# Autodesk Inventor assembly: ASM X-Axis
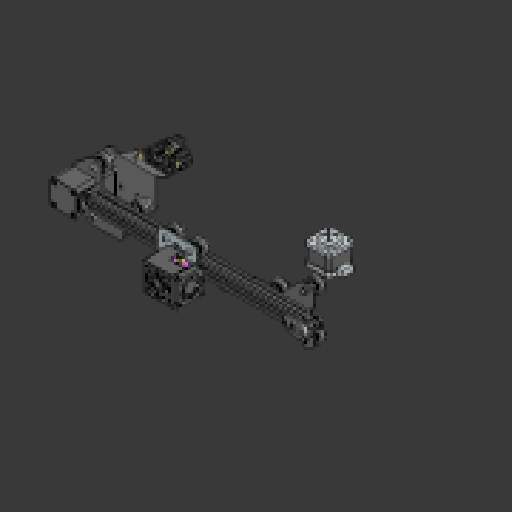
[picture p0: Inventor's stored thumbnail of the model, 512x512]
Saved by Autodesk Inventor 2023 (Build 270158000, 158)
## iProperties
Created: 2018-08-14
Part Number: ASM X-Axis
Document SubType Name: Assembly
Designer: alber
Sending System: SolidWorks 2015
Last Author: Poseidon
Last Saved: 2018-08-17
Author: alber
## Documents named in this file (26)
- C:\Users\alber\Desktop\Files\Ender3-Upgrade\CAD\ASM X-Axis.iam
- C:\Users\alber\Desktop\Files\Ender3-Upgrade\CAD\2020 profile.ipt
- C:\Users\alber\Desktop\Files\Ender3-Upgrade\CAD\Z Stent.ipt
- C:\Users\alber\Desktop\Files\Ender3-Upgrade\CAD\X motor bracket.ipt
- C:\Users\alber\Desktop\Files\Ender3-Upgrade\CAD\42-34 motor.ipt
- C:\Users\alber\Desktop\Files\Ender3-Upgrade\CAD\z nut.ipt
- C:\Users\alber\Desktop\Files\Ender3-Upgrade\CAD\E motor bracket.ipt
- C:\Users\alber\Desktop\Files\Ender3-Upgrade\CAD\X limit switch bracket.ipt
- C:\Users\alber\Desktop\Files\Ender3-Upgrade\CAD\X belt.ipt
- C:\Users\alber\Desktop\Files\Ender3-Upgrade\CAD\limit switch.ipt
- C:\Users\alber\Desktop\Files\Ender3-Upgrade\CAD\2GT-pulley.ipt
- C:\Users\alber\Desktop\Files\Ender3-Upgrade\CAD\Copper cover.ipt
- C:\Users\alber\Desktop\Files\Ender3-Upgrade\CAD\M4 Split Washer.ipt
- C:\Users\alber\Desktop\Files\Ender3-Upgrade\CAD\M3 Split Washer.ipt
- C:\Users\alber\Desktop\Files\Ender3-Upgrade\CAD\M4X16 Pan Head Screw.ipt
- C:\Users\alber\Desktop\Files\Ender3-Upgrade\CAD\M3X40-P.ipt
- C:\Users\alber\Desktop\Files\Ender3-Upgrade\CAD\M3X10 Pan Head Screw.ipt
- C:\Users\alber\Desktop\Files\Ender3-Upgrade\CAD\M3X6Pan Head Screw.ipt
- C:\Users\alber\Desktop\Files\Ender3-Upgrade\CAD\ASM Eccentrical Roller Z-Axis Left.iam
- C:\Users\alber\Desktop\Files\Ender3-Upgrade\CAD\ASM Roller Z-Axis Left.iam
- C:\Users\alber\Desktop\Files\Ender3-Upgrade\CAD\ASM Extruder.iam
- C:\Users\alber\Desktop\Files\Ender3-Upgrade\CAD\ASM X-Belt Tensioner.iam
- C:\Users\alber\Desktop\Files\Ender3-Upgrade\CAD\ASM Eccentrical Roller Z-Axis Right.iam
- C:\Users\alber\Desktop\Files\Ender3-Upgrade\CAD\ASM Roller Z-Axis Right.iam
- C:\Users\alber\Desktop\Files\Ender3-Upgrade\CAD\ASM Printing Head.iam
- C:\Users\alber\Desktop\Files\Ender3-Upgrade\CAD\Bowden_Tube.ipt
## Components (41 placed, 26 different names)
1. 2020 profile:1
2. Z Stent:1
3. X motor bracket:1
4. 42-34 motor:1
5. z nut:1
6. E motor bracket:1
7. X limit switch bracket:1
8. X belt:1
9. limit switch:1
10. 2GT-pulley:1
11. Copper cover:1
12. Copper cover:2
13. M4 Split Washer:2
14. M4 Split Washer:1
15. M3 Split Washer:1
16. M4X16 Pan Head Screw:1
17. M3X40-P:1
18. M4X16 Pan Head Screw:2
19. M3X40-P:2
20. M3X40-P:3
21. M3X40-P:4
22. M4X16 Pan Head Screw:4
23. M4 Split Washer:4
24. M4X16 Pan Head Screw:5
25. M4 Split Washer:5
26. M3X10 Pan Head Screw:3
27. M3 Split Washer:2
28. M3X10 Pan Head Screw:4
29. M3X6Pan Head Screw:1
30. M3X6Pan Head Screw:2
31. ASM Eccentrical Roller Z-Axis Left:1 [sub-assembly]
32. ASM Roller Z-Axis Left:1 [sub-assembly]
33. ASM Roller Z-Axis Left:2 [sub-assembly]
34. ASM Extruder:1 [sub-assembly] — Insert:1
35. ASM X-Belt Tensioner:1 [sub-assembly]
36. ASM Eccentrical Roller Z-Axis Right:1 [sub-assembly]
37. ASM Roller Z-Axis Right:1 [sub-assembly]
38. ASM Roller Z-Axis Right:2 [sub-assembly]
39. ASM Printing Head:1 [sub-assembly] — Flush:1
40. Extruder motor:2 — Insert:1
41. Bowden_Tube:1 — Flush:1
## Relationships (2: Insert 1, Flush 1)
- Insert:1: ASM Extruder:1 ↔ Extruder motor:2
- Flush:1: ASM Printing Head:1 ↔ Bowden_Tube:1
